# Autodesk Inventor assembly: updated table+legs
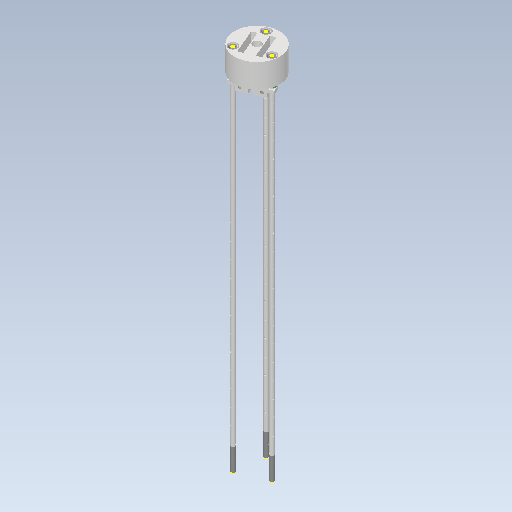
[picture p0: Inventor's stored thumbnail of the model, 512x512]
Saved by Autodesk Inventor 2020 (Build 240168000, 168)
## iProperties
Created: 2019-06-14
Part Number: updated table+legs
Document SubType Name: Assembly
Designer: ColinP
Mass: 19.4977 g
Surface Area: 238.161 cm^2
Volume: 19.4977 cm^3
Density: 1 g/cm^3
Author: ColinP
## Documents named in this file (8)
- C:\Users\ColinP\Documents\Inventor\ebeamheater v1\updated table+legs.iam
- C:\Users\ColinP\Documents\Inventor\ebeamheater v1\table.ipt
- C:\Users\ColinP\Documents\Inventor\ebeamheater v1\eyelet.ipt
- C:\Users\ColinP\Documents\Inventor\ebeamheater v1\assembly of 13 and 2.iam
- C:\Users\ColinP\Documents\Inventor\ebeamheater v1\washer.ipt
- C:\Users\ColinP\Documents\Inventor\ebeamheater v1\square eyelet.ipt
- C:\Users\ColinP\Documents\Inventor\ebeamheater v1\filament holders.ipt
- C:\Users\ColinP\Documents\Inventor\Content Center Files\R2020\en-US\ISO 4032(2)\ISO 4032 - M3 - ISO.ipt
## Components (18 placed, 7 different names)
1. table:1 — Insert:1, Insert:3, Insert:5, Insert:18, Insert:19, Insert:20, Angle:1, Angle:2
2. eyelet:1 — Insert:1, Insert:13
3. eyelet:3 — Insert:5, Insert:12
4. eyelet:4 — Insert:3, Insert:14
5. assembly of 13 and 2:1 [sub-assembly] — Insert:13, Insert:15, Insert:21
6. assembly of 13 and 2:2 [sub-assembly] — Insert:12, Insert:16
7. assembly of 13 and 2:3 [sub-assembly] — Insert:14, Insert:17, Insert:22
8. washer:1 — Insert:15, Insert:26
9. washer:2 — Insert:16, Insert:25
10. washer:3 — Insert:17, Insert:24
11. square eyelet:1 — Insert:19
12. square eyelet:2 — Insert:20
13. square eyelet:3 — Insert:18
14. filament holders:1 — Insert:21, Angle:1
15. filament holders:2 — Insert:22, Angle:2
16. ISO 4032 M3:1 — Insert:24
17. ISO 4032 M3:2 — Insert:25
18. ISO 4032 M3:3 — Insert:26
## Relationships (19: Insert 17, Angle 2)
- Insert:1: table:1 ↔ eyelet:1
- Insert:3: table:1 ↔ eyelet:4
- Insert:5: table:1 ↔ eyelet:3
- Insert:12 (-4.064 mm): eyelet:3 ↔ assembly of 13 and 2:2
- Insert:13 (-4.064 mm): eyelet:1 ↔ assembly of 13 and 2:1
- Insert:14 (-4.064 mm): eyelet:4 ↔ assembly of 13 and 2:3
- Insert:15 (-2.286 mm): assembly of 13 and 2:1 ↔ washer:1
- Insert:16 (-2.286 mm): assembly of 13 and 2:2 ↔ washer:2
- Insert:17 (-2.286 mm): assembly of 13 and 2:3 ↔ washer:3
- Insert:18: table:1 ↔ square eyelet:3
- Insert:19: table:1 ↔ square eyelet:1
- Insert:20: table:1 ↔ square eyelet:2
- Insert:21 (2.54 mm): assembly of 13 and 2:1 ↔ filament holders:1
- Insert:22 (2.54 mm): assembly of 13 and 2:3 ↔ filament holders:2
- Insert:24: washer:3 ↔ ISO 4032 M3:1
- Insert:25: washer:2 ↔ ISO 4032 M3:2
- Insert:26: washer:1 ↔ ISO 4032 M3:3
- Angle:1 (180 deg): table:1 ↔ filament holders:1
- Angle:2 (180 deg): table:1 ↔ filament holders:2
